# Autodesk Inventor assembly: アームアセンブリ2
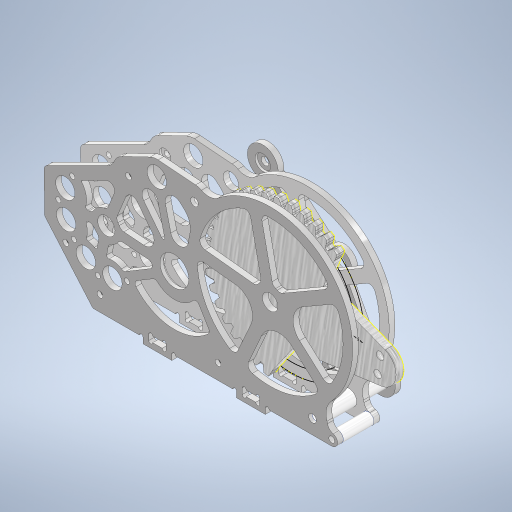
[picture p0: Inventor's stored thumbnail of the model, 512x512]
Saved by Autodesk Inventor 2023 (Build 270158000, 158)
## iProperties
Created: 2022-06-19
Part Number: アームアセンブリ2
Document SubType Name: Assembly
Designer: muzho
Author: muzho
## Documents named in this file (7)
- C:\Users\muzho\Documents\srdc\srdc_2\アーム\アームアセンブリ2.iam
- C:\Users\muzho\Documents\srdc\srdc_2\アーム\主フレーム.ipt
- C:\Users\muzho\Documents\srdc\srdc_2\アーム\右フレーム.ipt
- C:\Users\muzho\Documents\srdc\srdc_2\アーム(世古)\既製品\スペーサーm4-35　簡易筒型.ipt
- C:\Users\muzho\Documents\srdc\srdc_2\アーム(世古)\既製品\スペーサーm3-16　簡易筒型.ipt
- C:\Users\muzho\Documents\srdc\srdc_2\アーム\左フレーム.ipt
- C:\Users\muzho\Documents\srdc\srdc_2\アーム\ギア\最終段m2z40.ipt
## Components (6 placed, 6 different names)
1. 主フレーム:1 — メイト:1, メイト:2, 挿入:3, メイト:3, メイト:4
2. 右フレーム:1 — メイト:1, メイト:2, 挿入:1, 挿入:2, メイト:5
3. スペーサーm3-16　簡易筒型:1 — 挿入:1, 挿入:3
4. スペーサーm4-35　簡易筒型:1 — 挿入:2, 挿入:4
5. 左フレーム:1 — メイト:3, メイト:4, 挿入:4
6. 最終段m2z40:1 — メイト:5
## Relationships (9: Mate 5, Insert 4)
- メイト:1 [Mate]: 主フレーム:1 ↔ 右フレーム:1
- メイト:2 [Mate]: 主フレーム:1 ↔ 右フレーム:1
- 挿入:1 [Insert]: 右フレーム:1 ↔ スペーサーm3-16　簡易筒型:1
- 挿入:2 [Insert]: 右フレーム:1 ↔ スペーサーm4-35　簡易筒型:1
- 挿入:3 [Insert]: 主フレーム:1 ↔ スペーサーm3-16　簡易筒型:1
- メイト:3 [Mate]: 主フレーム:1 ↔ 左フレーム:1
- メイト:4 [Mate]: 主フレーム:1 ↔ 左フレーム:1
- 挿入:4 [Insert]: スペーサーm4-35　簡易筒型:1 ↔ 左フレーム:1
- メイト:5 [Mate]: 右フレーム:1 ↔ 最終段m2z40:1
